# Autodesk Inventor assembly: BBM Jig Assembly
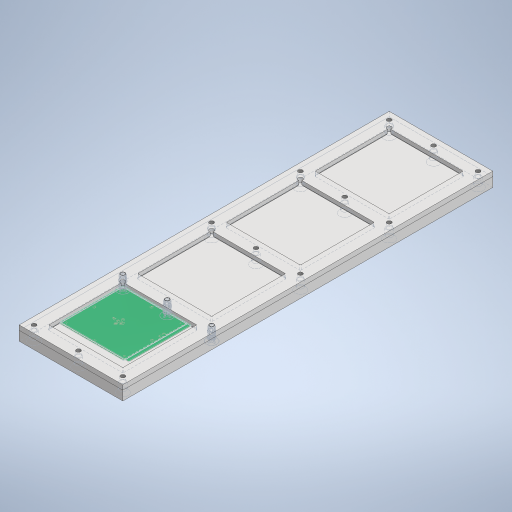
[picture p0: Inventor's stored thumbnail of the model, 512x512]
Saved by Autodesk Inventor 2023 (Build 270158000, 158)
## iProperties
Created: 2022-10-25
Part Number: BBM Jig Assembly
Document SubType Name: Assembly
Designer: Caleb
Author: Caleb
## Documents named in this file (6)
- C:\Users\Caleb\Desktop\nebraska-silicon-lab\Hardware\ETL\modules\throughput mockups\BBM Jig\BBM Jig Assembly.iam
- C:\Users\Caleb\Desktop\nebraska-silicon-lab\Hardware\ETL\modules\throughput mockups\BBM Jig\BBM Jig Base.ipt
- C:\Users\Caleb\Desktop\nebraska-silicon-lab\Hardware\ETL\modules\throughput mockups\BBM Jig\BBM Jig.ipt
- C:\Users\Caleb\Desktop\nebraska-silicon-lab\Hardware\ETL\modules\throughput mockups\throughput mockups\etl_lgad_mockup_v1p1.ipt
- C:\Users\Caleb\Desktop\nebraska-silicon-lab\Hardware\ETL\modules\throughput mockups\throughput mockups\etl_etroc_mockup_v1p1.ipt
- C:\Users\Caleb\Desktop\nebraska-silicon-lab\Hardware\ETL\modules\throughput mockups\BBM Jig\91771A065_Passivated 18-8 Stainless Steel Phillips Flat Head Screw.ipt
## Components (7 placed, 5 different names)
1. BBM Jig Base:1 — Mate:1, Flush:1, Flush:2, Mate:2, Insert:1, Insert:2, Insert:3
2. BBM Jig:1 — Mate:1, Flush:1, Flush:2, Mate:3, Mate:4, Mate:6, Mate:7
3. etl_lgad_mockup_v1p1:1 — Mate:2, Mate:3, Mate:4, Mate:5
4. etl_etroc_mockup_v1p1:1 — Mate:5, Mate:6, Mate:7
5. 91771A065_Passivated 18-8 Stainless Steel Phillips Flat Head Screw:1 — Insert:1
6. 91771A065_Passivated 18-8 Stainless Steel Phillips Flat Head Screw:2 — Insert:2
7. 91771A065_Passivated 18-8 Stainless Steel Phillips Flat Head Screw:3 — Insert:3
## Relationships (12: Mate 7, Insert 3, Flush 2)
- Mate:1: BBM Jig Base:1 ↔ BBM Jig:1
- Flush:1: BBM Jig Base:1 ↔ BBM Jig:1
- Flush:2: BBM Jig Base:1 ↔ BBM Jig:1
- Mate:2: BBM Jig Base:1 ↔ etl_lgad_mockup_v1p1:1
- Mate:3: BBM Jig:1 ↔ etl_lgad_mockup_v1p1:1
- Mate:4: BBM Jig:1 ↔ etl_lgad_mockup_v1p1:1
- Mate:5: etl_lgad_mockup_v1p1:1 ↔ etl_etroc_mockup_v1p1:1
- Mate:6: BBM Jig:1 ↔ etl_etroc_mockup_v1p1:1
- Mate:7: BBM Jig:1 ↔ etl_etroc_mockup_v1p1:1
- Insert:1: BBM Jig Base:1 ↔ 91771A065_Passivated 18-8 Stainless Steel Phillips Flat Head Screw:1
- Insert:2: BBM Jig Base:1 ↔ 91771A065_Passivated 18-8 Stainless Steel Phillips Flat Head Screw:2
- Insert:3: BBM Jig Base:1 ↔ 91771A065_Passivated 18-8 Stainless Steel Phillips Flat Head Screw:3
